# Autodesk Inventor assembly: ParallelMechanismus_Support_Rillenkugellager
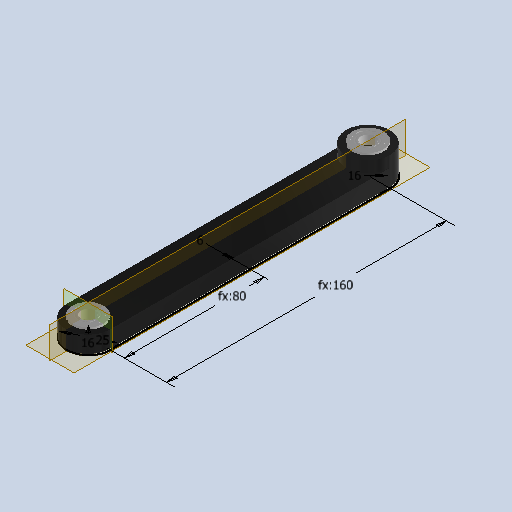
[picture p0: Inventor's stored thumbnail of the model, 512x512]
Saved by Autodesk Inventor 2024 (Build 280153000, 153)
## iProperties
Created: 2022-07-30
Part Number: ParallelMechanismus_Support_Rillenkugellager
Document SubType Name: Assembly
Designer: alexw
Mass: 67.8894 g
Surface Area: 183.917 cm^2
Volume: 44.3196 cm^3
Anlaufscheibe_JTM_1018_Dicke: 1,000 mm
Author: alexw
## Documents named in this file (3)
- C:\Users\AEWALDER\Documents\Inventor\03_CurrentProjects\MasterThesis\PSM_V1_Rillenkugellager\ParallelMechanismus_Support_Rillenkugellager.iam
- C:\Users\AEWALDER\Documents\Inventor\03_CurrentProjects\MasterThesis\PSM_V1_Rillenkugellager\ParallelSystem_ProximalPart_SupportLink.ipt
- C:\Users\AEWALDER\Documents\Inventor\03_CurrentProjects\MasterThesis\PSM_V1_Rillenkugellager\Maschinenbauteil\SKF_W 628_8 R-2RS1\SKF_W 628_8 R-2RS1.iam
## Components (4 placed, 2 different names)
1. ParallelSystem_ProximalPart_SupportLink:1 — Fluchtend:1, Fluchtend:2, Fluchtend:3, Passend:1, Passend:2, Passend:3, Passend:4, Passend:7, Passend:8
2. SKF_W 628_8 R-2RS1:1 [sub-assembly] — Passend:1, Passend:2
3. SKF_W 628_8 R-2RS1:2 [sub-assembly] — Passend:3, Passend:4
4. SKF_W 628_8 R-2RS1:3 [sub-assembly] — Passend:7, Passend:8
## Relationships (9: Mate 6, Flush 3)
- Fluchtend:1 [Flush]: ParallelSystem_ProximalPart_SupportLink:1
- Fluchtend:2 [Flush]: ParallelSystem_ProximalPart_SupportLink:1
- Fluchtend:3 [Flush]: ParallelSystem_ProximalPart_SupportLink:1
- Passend:1 [Mate]: ParallelSystem_ProximalPart_SupportLink:1 ↔ SKF_W 628_8 R-2RS1:1
- Passend:2 [Mate]: ParallelSystem_ProximalPart_SupportLink:1 ↔ SKF_W 628_8 R-2RS1:1
- Passend:3 [Mate]: ParallelSystem_ProximalPart_SupportLink:1 ↔ SKF_W 628_8 R-2RS1:2
- Passend:4 [Mate]: ParallelSystem_ProximalPart_SupportLink:1 ↔ SKF_W 628_8 R-2RS1:2
- Passend:7 [Mate]: ParallelSystem_ProximalPart_SupportLink:1 ↔ SKF_W 628_8 R-2RS1:3
- Passend:8 [Mate]: ParallelSystem_ProximalPart_SupportLink:1 ↔ SKF_W 628_8 R-2RS1:3
## Named parameters: Anlaufscheibe_JTM_1018_Dicke = 1 mm
